# Autodesk Inventor assembly: TestChamber
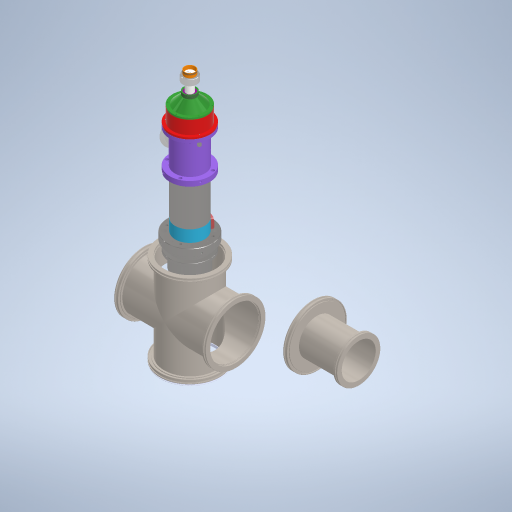
[picture p0: Inventor's stored thumbnail of the model, 512x512]
Saved by Autodesk Inventor 2023 (Build 270158000, 158)
## iProperties
Created: 2022-04-21
Part Number: TestChamber
Document SubType Name: Assembly
Designer: vmiguel
Author: vmiguel
## Documents named in this file (5)
- P:\SEM-Mechanical\TestChamber.iam
- P:\SEM-Mechanical\Hositrad_ISOX4-160.iam
- P:\SEM-Mechanical\Collumn.iam
- P:\SEM-Mechanical\Hositrad_ISO100-160R.iam
- P:\SEM-Mechanical\Hositrad_ISO160AV.ipt
## Components (4 placed, 4 different names)
1. Hositrad_ISOX4-160:1 [sub-assembly] — Rotational:1, Mate:1
2. Collumn:1 [sub-assembly] — Rotational:1
3. Hositrad_ISO100-160R:1 [sub-assembly]
4. Hositrad_ISO160AV:1 — Mate:1
## Relationships (2: RevoluteJoint 1, Mate 1)
- Rotational:1 [RevoluteJoint] (-10 mm): Hositrad_ISOX4-160:1 ↔ Collumn:1
- Mate:1: Hositrad_ISOX4-160:1 ↔ Hositrad_ISO160AV:1
